# Autodesk Inventor assembly: 4208K224_AIR CYLINDER
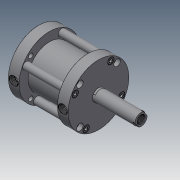
[picture p0: Inventor's stored thumbnail of the model, 180x180]
Saved by Autodesk Inventor 2018.3 (Build 223284000, 284)
## iProperties
Created: 2019-10-28
Vendor: HHMI: JRC - ID&F
Document SubType Name: Assembly
Designer: arnoldj
RuleStatus: InUse
AfterDocSave0: file://Part Number Cleaner
DESIGN DEPARTMENT: HHMI: JRC - ID&F
ALTERED ITEM PART NUMBER: N/A
ALTERED ITEM VENDOR: N/A
ALTERED ITEM DESCRIPTION: N/A
Author: arnoldj
Revision Number: 0
## Documents named in this file (3)
- C:\_WORKSPACE\DATA\COMMON\McMaster\4208K224_AIR CYLINDER.iam
- C:\_WORKSPACE\DATA\COMMON\McMaster\MCMASTER 4208K224_AIR CYLINDER BASE.ipt
- C:\_WORKSPACE\DATA\COMMON\McMaster\MCMASTER 4208K224_AIR CYLINDER SHAFT.ipt
## Components (2 placed, 2 different names)
1. MCMASTER 4208K224_AIR CYLINDER BASE:1 — Mate:1, Flush:2
2. MCMASTER 4208K224_AIR CYLINDER SHAFT:1 — Mate:1, Flush:2
## Relationships (2: Mate 1, Flush 1)
- Mate:1: MCMASTER 4208K224_AIR CYLINDER BASE:1 ↔ MCMASTER 4208K224_AIR CYLINDER SHAFT:1
- Flush:2: MCMASTER 4208K224_AIR CYLINDER BASE:1 ↔ MCMASTER 4208K224_AIR CYLINDER SHAFT:1
